# Autodesk Inventor assembly: Pièce 22-24
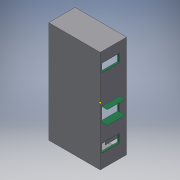
[picture p0: Inventor's stored thumbnail of the model, 180x180]
Saved by Autodesk Inventor 2016 SP1 (Build 200210100, 210)
## iProperties
Created: 2016-10-04
Part Number: Pièce 22-24
Material: Générique
Document SubType Name: Assembly
Designer: dimercur
DistanceMurBureau: 825,000 mm
Author: dimercur
## Documents named in this file (9)
- D:\Users\dimercur\Documents\SVN\projets-gei\Salle 22-24\Pièce 22-24.iam
- D:\Users\dimercur\Documents\SVN\projets-gei\Salle 22-24\Pièce.ipt
- D:\Users\dimercur\Documents\SVN\projets-gei\Salle 22-24\Fenetre.iam
- D:\Users\dimercur\Documents\SVN\projets-gei\Salle 22-24\Porte Simple.ipt
- D:\Users\dimercur\Documents\SVN\projets-gei\Salle 22-24\Porte Double.ipt
- D:\Users\dimercur\Documents\SVN\projets-gei\Salle 22-24\Poste de travail.iam
- D:\Users\dimercur\Documents\SVN\projets-gei\Salle 22-24\Poste de travail_MIR2.iam
- D:\Users\dimercur\Documents\SVN\projets-gei\Salle 22-24\Couvre-Radiateur.ipt
- D:\Users\dimercur\Documents\SVN\projets-gei\Salle 22-24\Ecran_Videoprojecteur.ipt
## Components (38 placed, 8 different names)
1. Pièce:1 — Placage:1, Placage:2, Placage:3, Placage:4, Placage:5, Placage:6, Placage:7, Placage:8, Placage:9, Placage:10, Placage:11, Placage:12, Placage:13, Placage:14, Placage:15, Placage:16, Placage:17, Placage:18, Affleurement:1, Placage:19, Placage:20, Placage:21, Placage:22, Placage:23, Placage:24
2. Porte Simple:1 — Placage:5, Placage:6, Placage:9
3. Porte Double:1 — Placage:4, Placage:7, Placage:8
4. Couvre-Radiateur:1 — Placage:14, Placage:15, Placage:16
5. Porte Simple:2 — Placage:17, Placage:18, Affleurement:1
6. Ecran_Videoprojecteur:1 — Placage:20, Placage:22, Placage:23
7. Ecran_Videoprojecteur:2 — Placage:19, Placage:21, Placage:24
8. Fenetre:1 [sub-assembly] — Placage:1, Placage:2, Placage:3
9. Fenetre:2 [sub-assembly]
10. Fenetre:3 [sub-assembly]
11. Fenetre:4 [sub-assembly]
12. Fenetre:5 [sub-assembly]
13. Fenetre:6 [sub-assembly]
14. Fenetre:7 [sub-assembly]
15. Poste de travail_MIR2:1 [sub-assembly]
16. Poste de travail:1 [sub-assembly] — Placage:11, Placage:12, Placage:13
17. Poste de travail_MIR2:2 [sub-assembly]
18. Poste de travail:2 [sub-assembly]
19. Poste de travail_MIR2:3 [sub-assembly]
20. Poste de travail:3 [sub-assembly]
21. Poste de travail_MIR2:4 [sub-assembly]
22. Poste de travail:4 [sub-assembly]
23. Poste de travail_MIR2:5 [sub-assembly]
24. Poste de travail:5 [sub-assembly]
25. Poste de travail_MIR2:6 [sub-assembly]
26. Poste de travail:6 [sub-assembly]
27. Poste de travail_MIR2:7 [sub-assembly]
28. Poste de travail:7 [sub-assembly]
29. Poste de travail_MIR2:8 [sub-assembly]
30. Poste de travail:8 [sub-assembly]
31. Poste de travail_MIR2:9 [sub-assembly]
32. Poste de travail:9 [sub-assembly]
33. Poste de travail_MIR2:10 [sub-assembly]
34. Poste de travail:10 [sub-assembly]
35. Poste de travail_MIR2:11 [sub-assembly]
36. Poste de travail:11 [sub-assembly]
37. Poste de travail_MIR2:12 [sub-assembly]
38. Poste de travail:12 [sub-assembly]
## Component patterns: (7 elements, first: Fenetre:1), (12 elements, first: Poste de travail_MIR2:1 + Poste de travail:1)
## Relationships (25: Mate 24, Flush 1)
- Placage:1 [Mate]: Pièce:1 ↔ Fenetre:1
- Placage:2 [Mate]: Pièce:1 ↔ Fenetre:1
- Placage:3 [Mate] (100 mm): Pièce:1 ↔ Fenetre:1
- Placage:4 [Mate]: Pièce:1 ↔ Porte Double:1
- Placage:5 [Mate]: Pièce:1 ↔ Porte Simple:1
- Placage:6 [Mate]: Pièce:1 ↔ Porte Simple:1
- Placage:7 [Mate]: Pièce:1 ↔ Porte Double:1
- Placage:8 [Mate]: Pièce:1 ↔ Porte Double:1
- Placage:9 [Mate]: Pièce:1 ↔ Porte Simple:1
- Placage:10 [Mate]: Pièce:1
- Placage:11 [Mate]: Pièce:1 ↔ Poste de travail:1
- Placage:12 [Mate]: Pièce:1 ↔ Poste de travail:1
- Placage:13 [Mate] (825 mm): Pièce:1 ↔ Poste de travail:1
- Placage:14 [Mate]: Pièce:1 ↔ Couvre-Radiateur:1
- Placage:15 [Mate]: Pièce:1 ↔ Couvre-Radiateur:1
- Placage:16 [Mate] (760 mm): Pièce:1 ↔ Couvre-Radiateur:1
- Placage:17 [Mate]: Pièce:1 ↔ Porte Simple:2
- Placage:18 [Mate]: Pièce:1 ↔ Porte Simple:2
- Affleurement:1 [Flush]: Pièce:1 ↔ Porte Simple:2
- Placage:19 [Mate]: Pièce:1 ↔ Ecran_Videoprojecteur:2
- Placage:20 [Mate]: Pièce:1 ↔ Ecran_Videoprojecteur:1
- Placage:21 [Mate] (700 mm): Pièce:1 ↔ Ecran_Videoprojecteur:2
- Placage:22 [Mate] (700 mm): Pièce:1 ↔ Ecran_Videoprojecteur:1
- Placage:23 [Mate] (1800 mm): Pièce:1 ↔ Ecran_Videoprojecteur:1
- Placage:24 [Mate] (2700 mm): Pièce:1 ↔ Ecran_Videoprojecteur:2
## Named parameters: DistanceMurBureau = 825 mm, EspaceEntreTravées = 2900 mm
